# Autodesk Inventor assembly: cam_holder_end_part_aligned
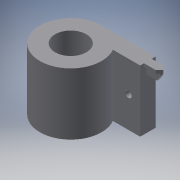
[picture p0: Inventor's stored thumbnail of the model, 180x180]
Saved by Autodesk Inventor 2019 (Build 230136000, 136)
## iProperties
Created: 2024-08-06
Part Number: cam_holder_end_part_aligned
Material: Generisch
Document SubType Name: Assembly
Designer: nic
Author: nic
## Documents named in this file (2)
- C:\Users\Nicolas Frick\Sync\OneDrive\wtm\nicol_rh8d\atxmega_qenc\inventor\cam_holder_end_part_aligned.iam
- C:\Users\Nicolas Frick\Sync\OneDrive\wtm\nicol_rh8d\atxmega_qenc\inventor\cam_holder_end_part.ipt
## Components (1 placed, 1 different names)
1. cam_holder_end_part:1 — Passend:1, Passend:2, Fluchtend:1, Fluchtend:2
## Relationships (4: Mate 2, Flush 2)
- Passend:1 [Mate]: cam_holder_end_part:1
- Passend:2 [Mate]: cam_holder_end_part:1
- Fluchtend:1 [Flush]: cam_holder_end_part:1
- Fluchtend:2 [Flush]: cam_holder_end_part:1
